# Autodesk Inventor assembly: top_cover
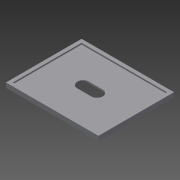
[picture p0: Inventor's stored thumbnail of the model, 180x180]
Saved by Autodesk Inventor 2014 SP1 (Build 180222100, 222)
## iProperties
Created: 2014-02-23
Part Number: top_cover
Document SubType Name: Assembly
Designer: Chris
Mass: 2436.34 g
Surface Area: 5824 cm^2
Volume: 2436.34 cm^3
Density: 1 g/cm^3
Author: Chris
## Documents named in this file (4)
- C:\Users\Chris\Documents\projects\langstroth_plain\inner_cover\inner_cover.iam
- C:\Users\Chris\Documents\projects\langstroth_plain\inner_cover\inner_cover_end.ipt
- C:\Users\Chris\Documents\projects\langstroth_plain\inner_cover\inner_cover_side.ipt
- C:\Users\Chris\Documents\projects\langstroth_plain\inner_cover\inner_cover_sheet.ipt
## Components (5 placed, 3 different names)
1. inner_cover_end:1 — Mate:3, Mate:7, Flush:1, Flush:5, Flush:6
2. inner_cover_end:2 — Mate:4, Mate:8, Flush:2, Flush:3, Flush:4
3. inner_cover_side:1 — Mate:2, Mate:5, Flush:1, Flush:2, Flush:6
4. inner_cover_side:2 — Mate:1, Mate:6, Flush:3, Flush:4, Flush:5
5. inner_cover_sheet:1 — Mate:1, Mate:2, Mate:3, Mate:4, Mate:5, Mate:6, Mate:7, Mate:8
## Relationships (14: Mate 8, Flush 6)
- Mate:1: inner_cover_side:2 ↔ inner_cover_sheet:1
- Mate:2: inner_cover_side:1 ↔ inner_cover_sheet:1
- Mate:3: inner_cover_end:1 ↔ inner_cover_sheet:1
- Mate:4: inner_cover_end:2 ↔ inner_cover_sheet:1
- Mate:5: inner_cover_side:1 ↔ inner_cover_sheet:1
- Mate:6: inner_cover_side:2 ↔ inner_cover_sheet:1
- Mate:7: inner_cover_end:1 ↔ inner_cover_sheet:1
- Mate:8: inner_cover_end:2 ↔ inner_cover_sheet:1
- Flush:1: inner_cover_end:1 ↔ inner_cover_side:1
- Flush:2: inner_cover_end:2 ↔ inner_cover_side:1
- Flush:3: inner_cover_end:2 ↔ inner_cover_side:2
- Flush:4: inner_cover_end:2 ↔ inner_cover_side:2
- Flush:5: inner_cover_end:1 ↔ inner_cover_side:2
- Flush:6: inner_cover_end:1 ↔ inner_cover_side:1
